# Autodesk Inventor assembly: assembly
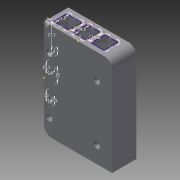
[picture p0: Inventor's stored thumbnail of the model, 180x180]
Saved by Autodesk Inventor 2015 (Build 190159000, 159)
## iProperties
Created: 2015-03-25
Part Number: assembly
Document SubType Name: Assembly
Designer: Pablo
Author: Pablo
## Documents named in this file (3)
- C:\programming\domocracy\dev\hub\Raspi\case\assembly.iam
- C:\programming\domocracy\dev\hub\Raspi\case\bottom.ipt
- C:\programming\domocracy\dev\hub\Raspi\case\top.ipt
## Components (2 placed, 2 different names)
1. bottom:1 — Mate:1, Flush:1, Flush:2
2. top:1 — Mate:1, Flush:1, Flush:2
## Relationships (3: Flush 2, Mate 1)
- Mate:1: bottom:1 ↔ top:1
- Flush:1: bottom:1 ↔ top:1
- Flush:2: bottom:1 ↔ top:1
